# Autodesk Inventor assembly: Assembly6
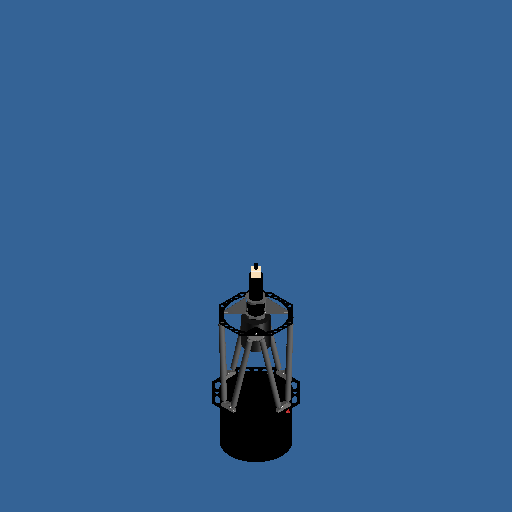
[picture p0: Inventor's stored thumbnail of the model, 512x512]
Saved by Autodesk Inventor 2026.2 (Build 302298000, 298)
## iProperties
Created: 2025-12-09
Part Number: Assembly6
Document SubType Name: Assembly
Designer: Thoma
Mass: 27295.5 g
Surface Area: 25498 cm^2
Volume: 10830.6 cm^3
Density: 2.52023 g/cm^3
Author: Thoma
## Documents named in this file (14)
- C:\Users\Thoma\OneDrive\Desktop\dir\telescope_cover\main\version_2\Main_v4.iam
- C:\Users\Thoma\OneDrive\Desktop\dir\telescope_cover\telescope\version_3\Telescope_End.ipt
- C:\Users\Thoma\OneDrive\Desktop\dir\telescope_cover\telescope\version_3\Triangle.ipt
- C:\Users\Thoma\OneDrive\Desktop\dir\telescope_cover\telescope\version_3\Triangle_Bracket_Top.ipt
- C:\Users\Thoma\OneDrive\Desktop\dir\telescope_cover\telescope\version_3\Carbon_Fibre.ipt
- C:\Users\Thoma\OneDrive\Desktop\dir\telescope_cover\telescope\version_3\5mm Screw.ipt
- C:\Users\Thoma\OneDrive\Desktop\dir\telescope_cover\telescope\version_3\35mm_bolt.ipt
- C:\Users\Thoma\OneDrive\Desktop\dir\telescope_cover\telescope\version_3\Triangle_Bracket_Bottom_MIR.ipt
- C:\Users\Thoma\OneDrive\Desktop\dir\telescope_cover\telescope\version_3\Telescope_Base.ipt
- C:\Users\Thoma\OneDrive\Desktop\dir\telescope_cover\telescope\version_3\Full_shaft_Simplify_3.ipt
- C:\Users\Thoma\OneDrive\Desktop\dir\telescope_cover\telescope\version_3\30mm_bolt.ipt
- C:\Users\Thoma\OneDrive\Desktop\dir\telescope_cover\telescope\version_3\Baffle.ipt
- C:\Users\Thoma\OneDrive\Desktop\dir\telescope_cover\telescope\version_3\Bottom_End_Top.ipt
- C:\Users\Thoma\OneDrive\Desktop\dir\telescope_cover\telescope\version_3\Laser.ipt
## Components (49 placed, 13 different names)
1. Laser:2 — Mate:214, Flush:220, Flush:221
2. Laser:1 — Mate:215, Flush:218, Flush:219
3. Baffle:1 — Mate:83
4. Carbon_Fibre:1 — Mate:7, Mate:11, Flush:1, Mate:12, Mate:13, Mate:14, Mate:15, Mate:62, Mate:83, Mate:92, Mate:93, Mate:96, Mate:97, Mate:98, Mate:100, Mate:123, Mate:124, Mate:125, Mate:213
5. Telescope_Base:1 — Mate:62, Angle:31, Mate:89, Mate:90, Angle:40, Mate:108, Mate:109, Angle:48, Mate:110, Mate:111, Angle:49, Mate:112, Mate:113, Angle:50, Mate:214, Mate:215, Flush:218, Flush:221
6. Telescope_End:1 — Mate:1, Mate:2, Angle:2, Mate:7, Mate:54, Mate:55, Angle:26, Angle:31, Mate:86, Mate:88, Mate:91, Angle:41, Mate:101, Angle:45, Angle:46, Mate:114, Mate:115, Angle:51, Mate:116, Mate:117, Angle:52, Mate:118, Mate:119, Angle:53
7. 30mm_bolt:9 — Mate:217, Mate:218, Angle:83
8. 30mm_bolt:10 — Mate:216, Mate:219, Angle:82
9. Triangle_Bracket_Top:5 — Mate:116, Mate:117, Angle:52, Mate:129, Flush:110, Angle:60
10. Triangle_Bracket_Top:4 — Mate:101, Angle:45, Angle:46, Mate:104, Mate:105, Mate:106, Flush:103, Angle:47
11. Triangle_Bracket_Top:3 — Mate:86, Mate:88, Mate:94, Angle:54, Angle:55, Mate:122, Flush:106, Angle:56
12. Triangle_Bracket_Top:1 — Mate:1, Mate:2, Angle:2, Mate:8, Mate:9, Angle:4, Mate:47, Angle:22, Mate:58
13. Triangle:1 — Mate:8, Mate:9, Angle:4, Mate:11, Flush:1, Angle:5, Angle:6, Mate:46
14. Triangle:5 — Mate:92, Mate:93, Mate:94, Mate:128, Flush:109, Angle:59, Flush:181, Angle:81
15. Triangle:6 — Mate:96, Mate:97, Mate:98, Flush:102, Angle:44, Mate:104, Mate:105
16. Triangle:7 — Mate:123, Mate:124, Mate:125, Mate:126, Flush:107, Angle:57, Mate:127, Flush:108, Angle:58
17. 35mm_bolt:6 — Mate:122, Flush:106, Angle:56
18. 35mm_bolt:7 — Mate:129, Flush:110, Angle:60
19. 35mm_bolt:4 — Mate:46, Mate:47, Angle:22
20. 35mm_bolt:5 — Mate:106, Flush:103, Angle:47
21. 5mm Screw:9 — Mate:100, Flush:102, Angle:44
22. 5mm Screw:13 — Mate:213, Flush:181, Angle:81
23. 5mm Screw:10 — Mate:126, Flush:107, Angle:57
24. 5mm Screw:2 — Mate:14, Mate:15, Angle:6
25. 5mm Screw:1 — Mate:12, Mate:13, Angle:5
26. 5mm Screw:11 — Mate:127, Flush:108, Angle:58
27. 5mm Screw:12 — Mate:128, Flush:109, Angle:59
28. Full_shaft_Simplify_3:1
29. Full_shaft_Simplify_3:2 — Tangent:26
30. Full_shaft_Simplify_3:3
31. Full_shaft_Simplify_3:4
32. Full_shaft_Simplify_3:5
33. Full_shaft_Simplify_3:6
34. Full_shaft_Simplify_3:7
35. Full_shaft_Simplify_3:8 — Tangent:31, Tangent:33
36. 30mm_bolt:7 — Mate:120, Flush:104, Angle:54
37. 30mm_bolt:1 — Mate:121, Flush:105, Angle:55
38. 30mm_bolt:8 — Mate:80, Flush:13, Angle:39
39. 30mm_bolt:6 — Mate:78, Flush:11, Angle:37
40. 30mm_bolt:3 — Mate:79, Flush:12, Angle:38
41. 30mm_bolt:2 — Mate:77, Flush:10, Angle:36
42. Triangle_Bracket_Bottom_MIR:4 — Mate:118, Mate:119, Angle:53, Mate:216, Mate:217, Mate:218, Mate:219, Angle:82, Angle:83
43. Triangle_Bracket_Bottom_MIR:3 — Mate:114, Mate:115, Angle:51, Mate:120, Flush:104, Mate:121, Flush:105
44. Triangle_Bracket_Bottom_MIR:2 — Mate:55, Mate:58, Angle:26, Mate:77, Flush:10, Angle:36, Mate:78, Flush:11, Angle:37, Tangent:31
45. Triangle_Bracket_Bottom_MIR:1 — Mate:54, Mate:79, Flush:12, Angle:38, Mate:80, Flush:13, Angle:39, Mate:91, Angle:41
46. Bottom_End_Top:4 — Mate:112, Mate:113, Angle:50, Tangent:26, Tangent:33
47. Bottom_End_Top:3 — Mate:110, Mate:111, Angle:49, Flush:219
48. Bottom_End_Top:2 — Mate:108, Mate:109, Angle:48
49. Bottom_End_Top:1 — Mate:89, Mate:90, Angle:40, Flush:220
## Relationships (121: Mate 66, Angle 33, Flush 19, Tangent 3)
- Mate:1: Telescope_End:1 ↔ Triangle_Bracket_Top:1
- Mate:2: Telescope_End:1 ↔ Triangle_Bracket_Top:1
- Angle:2 (0 deg): Telescope_End:1 ↔ Triangle_Bracket_Top:1
- Mate:7: Carbon_Fibre:1 ↔ Telescope_End:1
- Mate:8: Triangle_Bracket_Top:1 ↔ Triangle:1
- Mate:9: Triangle_Bracket_Top:1 ↔ Triangle:1
- Angle:4 (0 deg): Triangle_Bracket_Top:1 ↔ Triangle:1
- Mate:11: Carbon_Fibre:1 ↔ Triangle:1
- Flush:1: Carbon_Fibre:1 ↔ Triangle:1
- Mate:12: Carbon_Fibre:1 ↔ 5mm Screw:1
- Mate:13: Carbon_Fibre:1 ↔ 5mm Screw:1
- Angle:5 (0 deg): Triangle:1 ↔ 5mm Screw:1
- Mate:14: Carbon_Fibre:1 ↔ 5mm Screw:2
- Mate:15: Carbon_Fibre:1 ↔ 5mm Screw:2
- Angle:6 (0 deg): Triangle:1 ↔ 5mm Screw:2
- Mate:46: Triangle:1 ↔ 35mm_bolt:4
- Mate:47: Triangle_Bracket_Top:1 ↔ 35mm_bolt:4
- Angle:22 (0 deg): Triangle_Bracket_Top:1 ↔ 35mm_bolt:4
- Mate:54: Telescope_End:1 ↔ Triangle_Bracket_Bottom_MIR:1
- Mate:55: Telescope_End:1 ↔ Triangle_Bracket_Bottom_MIR:2
- Mate:58: Triangle_Bracket_Top:1 ↔ Triangle_Bracket_Bottom_MIR:2
- Angle:26 (0 deg): Telescope_End:1 ↔ Triangle_Bracket_Bottom_MIR:2
- Mate:62: Carbon_Fibre:1 ↔ Telescope_Base:1
- Angle:31 (0 deg): Telescope_Base:1 ↔ Telescope_End:1
- Mate:77: 30mm_bolt:2 ↔ Triangle_Bracket_Bottom_MIR:2
- Flush:10: 30mm_bolt:2 ↔ Triangle_Bracket_Bottom_MIR:2
- Angle:36 (0 deg): 30mm_bolt:2 ↔ Triangle_Bracket_Bottom_MIR:2
- Mate:78: 30mm_bolt:6 ↔ Triangle_Bracket_Bottom_MIR:2
- Flush:11: 30mm_bolt:6 ↔ Triangle_Bracket_Bottom_MIR:2
- Angle:37 (0 deg): 30mm_bolt:6 ↔ Triangle_Bracket_Bottom_MIR:2
- Mate:79: 30mm_bolt:3 ↔ Triangle_Bracket_Bottom_MIR:1
- Flush:12: 30mm_bolt:3 ↔ Triangle_Bracket_Bottom_MIR:1
- Angle:38 (0 deg): 30mm_bolt:3 ↔ Triangle_Bracket_Bottom_MIR:1
- Mate:80: 30mm_bolt:8 ↔ Triangle_Bracket_Bottom_MIR:1
- Flush:13: 30mm_bolt:8 ↔ Triangle_Bracket_Bottom_MIR:1
- Angle:39 (0 deg): 30mm_bolt:8 ↔ Triangle_Bracket_Bottom_MIR:1
- Mate:83: Baffle:1 ↔ Carbon_Fibre:1
- Mate:86: Telescope_End:1 ↔ Triangle_Bracket_Top:3
- Mate:88: Telescope_End:1 ↔ Triangle_Bracket_Top:3
- Mate:89: Telescope_Base:1 ↔ Bottom_End_Top:1
- Mate:90: Telescope_Base:1 ↔ Bottom_End_Top:1
- Angle:40 (0 deg): Telescope_Base:1 ↔ Bottom_End_Top:1
- Mate:91: Telescope_End:1 ↔ Triangle_Bracket_Bottom_MIR:1
- Angle:41 (0 deg): Telescope_End:1 ↔ Triangle_Bracket_Bottom_MIR:1
- Mate:92: Carbon_Fibre:1 ↔ Triangle:5
- Mate:93: Carbon_Fibre:1 ↔ Triangle:5
- Mate:94: Triangle_Bracket_Top:3 ↔ Triangle:5
- Mate:96: Carbon_Fibre:1 ↔ Triangle:6
- Mate:97: Carbon_Fibre:1 ↔ Triangle:6
- Mate:98: Carbon_Fibre:1 ↔ Triangle:6
- Mate:100: Carbon_Fibre:1 ↔ 5mm Screw:9
- Flush:102: Triangle:6 ↔ 5mm Screw:9
- Angle:44 (0 deg): Triangle:6 ↔ 5mm Screw:9
- Mate:101: Telescope_End:1 ↔ Triangle_Bracket_Top:4
- Angle:45 (0 deg): Telescope_End:1 ↔ Triangle_Bracket_Top:4
- Angle:46 (0 deg): Telescope_End:1 ↔ Triangle_Bracket_Top:4
- Mate:104: Triangle_Bracket_Top:4 ↔ Triangle:6
- Mate:105: Triangle_Bracket_Top:4 ↔ Triangle:6
- Mate:106: Triangle_Bracket_Top:4 ↔ 35mm_bolt:5
- Flush:103: Triangle_Bracket_Top:4 ↔ 35mm_bolt:5
- Angle:47 (0 deg): Triangle_Bracket_Top:4 ↔ 35mm_bolt:5
- Mate:108: Telescope_Base:1 ↔ Bottom_End_Top:2
- Mate:109: Telescope_Base:1 ↔ Bottom_End_Top:2
- Angle:48 (0 deg): Telescope_Base:1 ↔ Bottom_End_Top:2
- Mate:110: Telescope_Base:1 ↔ Bottom_End_Top:3
- Mate:111: Telescope_Base:1 ↔ Bottom_End_Top:3
- Angle:49 (0 deg): Telescope_Base:1 ↔ Bottom_End_Top:3
- Mate:112: Telescope_Base:1 ↔ Bottom_End_Top:4
- Mate:113: Telescope_Base:1 ↔ Bottom_End_Top:4
- Angle:50 (0 deg): Telescope_Base:1 ↔ Bottom_End_Top:4
- Mate:114: Telescope_End:1 ↔ Triangle_Bracket_Bottom_MIR:3
- Mate:115: Telescope_End:1 ↔ Triangle_Bracket_Bottom_MIR:3
- Angle:51 (0 deg): Telescope_End:1 ↔ Triangle_Bracket_Bottom_MIR:3
- Mate:116: Telescope_End:1 ↔ Triangle_Bracket_Top:5
- Mate:117: Telescope_End:1 ↔ Triangle_Bracket_Top:5
- Angle:52 (0 deg): Telescope_End:1 ↔ Triangle_Bracket_Top:5
- Mate:118: Telescope_End:1 ↔ Triangle_Bracket_Bottom_MIR:4
- Mate:119: Telescope_End:1 ↔ Triangle_Bracket_Bottom_MIR:4
- Angle:53 (0 deg): Telescope_End:1 ↔ Triangle_Bracket_Bottom_MIR:4
- Mate:120: 30mm_bolt:7 ↔ Triangle_Bracket_Bottom_MIR:3
- Flush:104: 30mm_bolt:7 ↔ Triangle_Bracket_Bottom_MIR:3
- Angle:54 (0 deg): Triangle_Bracket_Top:3 ↔ 30mm_bolt:7
- Mate:121: 30mm_bolt:1 ↔ Triangle_Bracket_Bottom_MIR:3
- Flush:105: 30mm_bolt:1 ↔ Triangle_Bracket_Bottom_MIR:3
- Angle:55 (0 deg): Triangle_Bracket_Top:3 ↔ 30mm_bolt:1
- Mate:122: Triangle_Bracket_Top:3 ↔ 35mm_bolt:6
- Flush:106: Triangle_Bracket_Top:3 ↔ 35mm_bolt:6
- Angle:56 (0 deg): Triangle_Bracket_Top:3 ↔ 35mm_bolt:6
- Mate:123: Carbon_Fibre:1 ↔ Triangle:7
- Mate:124: Carbon_Fibre:1 ↔ Triangle:7
- Mate:125: Carbon_Fibre:1 ↔ Triangle:7
- Mate:126: Triangle:7 ↔ 5mm Screw:10
- Flush:107: Triangle:7 ↔ 5mm Screw:10
- Angle:57 (0 deg): Triangle:7 ↔ 5mm Screw:10
- Mate:127: Triangle:7 ↔ 5mm Screw:11
- Flush:108: Triangle:7 ↔ 5mm Screw:11
- Angle:58 (0 deg): Triangle:7 ↔ 5mm Screw:11
- Mate:128: Triangle:5 ↔ 5mm Screw:12
- Flush:109: Triangle:5 ↔ 5mm Screw:12
- Angle:59 (0 deg): Triangle:5 ↔ 5mm Screw:12
- Mate:129: Triangle_Bracket_Top:5 ↔ 35mm_bolt:7
- Flush:110: Triangle_Bracket_Top:5 ↔ 35mm_bolt:7
- Angle:60 (0 deg): Triangle_Bracket_Top:5 ↔ 35mm_bolt:7
- Mate:213: Carbon_Fibre:1 ↔ 5mm Screw:13
- Flush:181: Triangle:5 ↔ 5mm Screw:13
- Angle:81 (0 deg): Triangle:5 ↔ 5mm Screw:13
- Mate:214: Laser:2 ↔ Telescope_Base:1
- Mate:215: Laser:1 ↔ Telescope_Base:1
- Flush:218: Laser:1 ↔ Telescope_Base:1
- Flush:219 (39.316 mm): Laser:1 ↔ Bottom_End_Top:3
- Flush:220 (39.316 mm): Laser:2 ↔ Bottom_End_Top:1
- Flush:221: Laser:2 ↔ Telescope_Base:1
- Tangent:26: Full_shaft_Simplify_3:2 ↔ Bottom_End_Top:4
- Tangent:31: Full_shaft_Simplify_3:8 ↔ Triangle_Bracket_Bottom_MIR:2
- Tangent:33: Full_shaft_Simplify_3:8 ↔ Bottom_End_Top:4
- Mate:216: 30mm_bolt:10 ↔ Triangle_Bracket_Bottom_MIR:4
- Mate:217: 30mm_bolt:9 ↔ Triangle_Bracket_Bottom_MIR:4
- Mate:218: 30mm_bolt:9 ↔ Triangle_Bracket_Bottom_MIR:4
- Mate:219: 30mm_bolt:10 ↔ Triangle_Bracket_Bottom_MIR:4
- Angle:82 (0 deg): 30mm_bolt:10 ↔ Triangle_Bracket_Bottom_MIR:4
- Angle:83 (0 deg): 30mm_bolt:9 ↔ Triangle_Bracket_Bottom_MIR:4
